# Autodesk Inventor assembly: printed carriage assembly
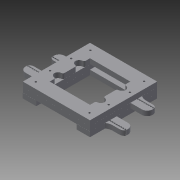
[picture p0: Inventor's stored thumbnail of the model, 180x180]
Saved by Autodesk Inventor 2014 SP1 (Build 180222100, 222)
## iProperties
Created: 2014-10-23
Part Number: printed carriage assembly
Document SubType Name: Assembly
Designer: Mon
Author: Mon
## Documents named in this file (3)
- H:\core xy\printed carriage assembly.iam
- H:\core xy\core xy carriage.ipt
- H:\core xy\x carriage belt tensioner.ipt
## Components (3 placed, 2 different names)
1. core xy carriage:1 — Mate:1
2. x carriage belt tensioner:1 — Mate:1, Mate:2
3. x carriage belt tensioner:2 — Mate:2
## Relationships (2: Mate 2)
- Mate:1: core xy carriage:1 ↔ x carriage belt tensioner:1
- Mate:2: x carriage belt tensioner:1 ↔ x carriage belt tensioner:2
